# Autodesk Inventor assembly: Assembly_Anglerfish_3inch_Tube_v0
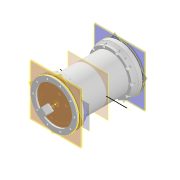
[picture p0: Inventor's stored thumbnail of the model, 180x180]
Saved by Autodesk Inventor 2022 (Build 260153000, 153)
## iProperties
Created: 2022-04-12
Part Number: Assembly_Anglerfish_3inch_Tube_v0
Document SubType Name: Assembly
Designer: Prakash Lab
Author: Prakash Lab
## Documents named in this file (12)
- C:\Users\PrakashLab\Documents\Matchboxscope\INVENTOR\Assembly_Anglerfish_3inch_Tube_v0.iam
- C:\Users\PrakashLab\Documents\Matchboxscope\INVENTOR\00_Tube_3inch.ipt
- C:\Users\PrakashLab\Documents\Matchboxscope\INVENTOR\Anglerfish_3inch_tube_endpiece.ipt
- C:\Users\PrakashLab\Documents\Matchboxscope\INVENTOR\Anglerfish_Frontwindow_3inchtube_V0.ipt
- C:\Users\PrakashLab\Documents\Matchboxscope\INVENTOR\Matchboxscope_middle2_v1.ipt
- C:\Users\PrakashLab\Documents\Matchboxscope\INVENTOR\Matchboxscope_Lightperiscope_V0.ipt
- C:\Users\PrakashLab\Documents\Matchboxscope\INVENTOR\Matchboxscope_bottom_v0.ipt
- C:\Users\PrakashLab\Documents\Matchboxscope\INVENTOR\00_ESP3-CAM.iam
- C:\Users\PrakashLab\Documents\Matchboxscope\INVENTOR\Matchboxscope_lenstube_v0.ipt
- C:\Users\PrakashLab\Documents\Matchboxscope\INVENTOR\00_Powerbank.ipt
- C:\Users\PrakashLab\Documents\Matchboxscope\INVENTOR\Anglerfish_3inch_tube_adapterplate_focus.ipt
- C:\Users\PrakashLab\Documents\Matchboxscope\INVENTOR\Anglerfish_3inch_tube_pressurering.ipt
## Components (14 placed, 11 different names)
1. Matchboxscope_middle2_v1:1 — Flush:5, Flush:6, Insert:3
2. Matchboxscope_bottom_v0:1
3. 00_ESP3-CAM:1 [sub-assembly]
4. 00_Powerbank:1
5. Anglerfish_3inch_tube_adapterplate_focus:1 — Flush:5, Flush:6, Mate:7, Flush:7, Insert:5
6. Matchboxscope_lenstube_v0:2 — Insert:3, Mate:8
7. Matchboxscope_Lightperiscope_V0:1 — Mate:7, Mate:8, Flush:7
8. 00_Tube_3inch:1 — Insert:7, Mate:10
9. Anglerfish_3inch_tube_endpiece:1 — Insert:6, Mate:9, Insert:7
10. Anglerfish_Frontwindow_3inchtube_V0:1 — Insert:5, Insert:6, Mate:9, Flush:8, Flush:9
11. Anglerfish_3inch_tube_pressurering:1 — Flush:8, Flush:9
12. Anglerfish_3inch_tube_endpiece:2
13. Anglerfish_Frontwindow_3inchtube_V0:2
14. Anglerfish_3inch_tube_pressurering:2
## Component patterns: (2 elements, first: Anglerfish_3inch_tube_endpiece:1 + Anglerfish_Frontwindow_3inchtube_V0:1 + Anglerfish_3inch_tube_pressurering:1)
## Relationships (20: Mate 9, Flush 6, Insert 5)
- [Mate]: Matchboxscope_bottom_v0:1 ↔ 00_ESP3-CAM:1
- [Flush]: Matchboxscope_bottom_v0:1 ↔ 00_ESP3-CAM:1
- [Insert]: Matchboxscope_middle2_v1:1 ↔ 00_ESP3-CAM:1
- [Mate]: Matchboxscope_middle2_v1:1 ↔ Matchboxscope_bottom_v0:1
- [Mate]: Matchboxscope_bottom_v0:1 ↔ 00_Powerbank:1
- [Mate]: Matchboxscope_bottom_v0:1 ↔ 00_Powerbank:1
- [Mate] (5 mm): Matchboxscope_bottom_v0:1 ↔ 00_Powerbank:1
- Flush:5: Matchboxscope_middle2_v1:1 ↔ Anglerfish_3inch_tube_adapterplate_focus:1
- Flush:6: Matchboxscope_middle2_v1:1 ↔ Anglerfish_3inch_tube_adapterplate_focus:1
- Insert:3: Matchboxscope_middle2_v1:1 ↔ Matchboxscope_lenstube_v0:2
- Mate:7: Anglerfish_3inch_tube_adapterplate_focus:1 ↔ Matchboxscope_Lightperiscope_V0:1
- Mate:8: Matchboxscope_lenstube_v0:2 ↔ Matchboxscope_Lightperiscope_V0:1
- Flush:7 (-30 mm): Anglerfish_3inch_tube_adapterplate_focus:1 ↔ Matchboxscope_Lightperiscope_V0:1
- Insert:5 (0.5 mm): Anglerfish_3inch_tube_adapterplate_focus:1 ↔ Anglerfish_Frontwindow_3inchtube_V0:1
- Insert:6: Anglerfish_3inch_tube_endpiece:1 ↔ Anglerfish_Frontwindow_3inchtube_V0:1
- Mate:9: Anglerfish_3inch_tube_endpiece:1 ↔ Anglerfish_Frontwindow_3inchtube_V0:1
- Insert:7: 00_Tube_3inch:1 ↔ Anglerfish_3inch_tube_endpiece:1
- Flush:8: Anglerfish_Frontwindow_3inchtube_V0:1 ↔ Anglerfish_3inch_tube_pressurering:1
- Flush:9: Anglerfish_Frontwindow_3inchtube_V0:1 ↔ Anglerfish_3inch_tube_pressurering:1
- Mate:10: 00_Tube_3inch:1
## Named parameters: d3_d8 = 0 mm
